# Autodesk Inventor assembly: chassis
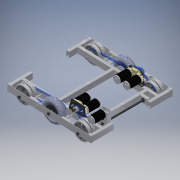
[picture p0: Inventor's stored thumbnail of the model, 180x180]
Saved by Autodesk Inventor 2016 (Build 200138000, 138)
## iProperties
Created: 2016-01-16
Part Number: chassis
Document SubType Name: Assembly
Designer: gus
Mass: 17272.6 g
Surface Area: 33201.5 cm^2
Volume: 7181.59 cm^3
Density: 2.40513 g/cm^3
Author: gus
## Documents named in this file (20)
- \\Mac\Home\Desktop\1510-stronghold-CAD\chassis\chassis.iam
- \\Mac\Home\Desktop\1510-stronghold-CAD\chassis\1x2x28.ipt
- \\Mac\Home\Desktop\1510-stronghold-CAD\chassis\1x2x19.ipt
- \\Mac\Home\Desktop\1510-stronghold-CAD\chassis\1x2x8in.ipt
- \\Mac\Home\Desktop\1510-stronghold-CAD\chassis\3 in churro.ipt
- \\Mac\Home\Desktop\1510-stronghold-CAD\chassis\side plate.ipt
- \\Mac\Home\Desktop\1510-stronghold-CAD\chassis\PneumaticWheel_am-0970-2.iam
- \\Mac\Home\Desktop\1510-stronghold-CAD\chassis\CIMple Box\CIMple Box.iam
- \\Mac\Home\Desktop\1510-stronghold-CAD\chassis\am-0736_S35-12DHE.ipt
- \\Mac\Home\Desktop\1510-stronghold-CAD\chassis\am-940a-6-HiGrip-.iam
- \\Mac\Home\Desktop\1510-stronghold-CAD\chassis\half-inch hex bolt.ipt
- \\Mac\Home\Desktop\1510-stronghold-CAD\chassis\half-inch hex nut.ipt
- \\Mac\Home\Desktop\1510-stronghold-CAD\chassis\wheel arm support.ipt
- \\Mac\Home\Desktop\1510-stronghold-CAD\roller wheels\toughbox micro\Toughbox+Nano+All+Shafts+v2-2.iam
- \\Mac\Home\Desktop\1510-stronghold-CAD\roller wheels\hex bearing.ipt
- \\Mac\Home\Desktop\1510-stronghold-CAD\chassis\chassis\Design Accelerator\Chain Drive13.iam
- \\Mac\Home\Desktop\1510-stronghold-CAD\chassis\chassis\Design Accelerator\Chain Drive14.iam
- \\Mac\Home\Desktop\1510-stronghold-CAD\chassis\chassis\Design Accelerator\Chain Drive15.iam
- \\Mac\Home\Desktop\1510-stronghold-CAD\chassis\chassis\Design Accelerator\Chain Drive16.iam
- \\Mac\Home\Desktop\1510-stronghold-CAD\chassis\chassis\Design Accelerator\Chain Drive17.iam
## Components (48 placed, 15 different names)
1. 1x2x28:1 — Mate:1, Mate:2, Flush:1, Flush:2, Mate:4, Flush:4, Flush:6, Flush:12, Flush:13, Mate:19, Rotational:7, Rotational:8, Cylindrical:25, Rotational:18, Rotational:29, Cylindrical:22, Mate:41, Flush:31, Mate:57, Mate:58
2. 1x2x19:1 — Mate:1, Flush:2, Mate:12, Mate:13, Flush:22
3. 1x2x19:2 — Mate:2, Flush:1, Mate:34, Flush:26, Flush:27, Flush:33, Mate:59, Mate:60
4. 1x2x8in:1 — Mate:8, Flush:10, Mate:13, Mate:35
5. 1x2x8in:2 — Mate:4, Flush:4, Flush:6, Mate:9, Flush:11, Mate:12, Mate:62
6. 3 in churro:1 — Mate:10, Flush:13, Flush:38
7. 3 in churro:2 — Mate:11, Flush:12, Flush:37
8. 3 in churro:3 — Flush:23, Mate:36, Flush:36
9. 3 in churro:4 — Flush:24, Mate:37, Flush:35
10. side plate:1 — Mate:8, Flush:10, Mate:21, Rotational:23, Rotational:24, Rotational:25, Mate:61
11. side plate:2 — Mate:9, Flush:11, Mate:10, Mate:11, Mate:22, Rotational:26, Rotational:27, Rotational:28, Mate:62
12. PneumaticWheel_am-0970-2:1 [sub-assembly] — Rotational:20, Flush:39, Flush:40
13. 1x2x8in:3 — Mate:19, Mate:22, Mate:53, Flush:34
14. 1x2x8in:4 — Mate:21, Mate:33, Flush:20, Flush:21, Flush:28, Mate:39, Mate:61
15. am-0736_S35-12DHE:1 — Cylindrical:2, Mate:49
16. am-0736_S35-12DHE:2 — Mate:50, Cylindrical:26
17. am-940a-6-HiGrip-:1 [sub-assembly] — Cylindrical:25, Flush:42
18. am-940a-6-HiGrip-:2 [sub-assembly] — Cylindrical:22, Flush:41
19. am-940a-6-HiGrip-:3 [sub-assembly] — Cylindrical:23, Flush:40
20. am-940a-6-HiGrip-:4 [sub-assembly] — Cylindrical:24, Flush:39
21. half-inch hex bolt:2 — Rotational:12
22. half-inch hex bolt:4 — Rotational:14
23. half-inch hex bolt:5 — Rotational:7
24. half-inch hex bolt:6 — Rotational:8
25. PneumaticWheel_am-0970-2:2 [sub-assembly] — Rotational:29, Flush:41, Flush:42
26. 1x2x28:2 — Mate:33, Flush:20, Mate:34, Flush:21, Mate:35, Flush:22, Flush:23, Flush:24, Mate:36, Mate:37, Rotational:12, Rotational:14, Cylindrical:24, Rotational:17, Rotational:20, Cylindrical:23, Mate:42, Flush:32, Mate:55, Mate:56
27. half-inch hex bolt:7 — Rotational:17
28. half-inch hex bolt:8 — Rotational:18
29. half-inch hex nut:1 — Rotational:23
30. half-inch hex nut:2 — Rotational:27
31. half-inch hex nut:3 — Rotational:25
32. half-inch hex nut:4 — Rotational:26
33. half-inch hex nut:5 — Rotational:28
34. half-inch hex nut:6 — Rotational:24
35. wheel arm support:1 — Flush:26, Flush:27, Flush:28, Mate:39, Rotational:30
36. CIMple Box:1 [sub-assembly] — Mate:41, Flush:31, Mate:50, Cylindrical:26, Mate:60
37. CIMple Box:2 [sub-assembly] — Mate:42, Flush:32, Cylindrical:2, Mate:49, Mate:59
38. Toughbox+Nano+All+Shafts+v2-2:1 [sub-assembly] — Flush:33, Mate:53, Flush:34, Mate:54
39. hex bearing:1 — Rotational:30, Mate:54
40. 3 in churro:5 — Mate:55, Flush:35
41. 3 in churro:6 — Mate:56, Flush:36
42. 3 in churro:7 — Mate:57, Flush:37
43. 3 in churro:8 — Mate:58, Flush:38
44. Chain Drive:1 [sub-assembly]
45. Chain Drive:2 [sub-assembly]
46. Chain Drive:3 [sub-assembly]
47. Chain Drive:4 [sub-assembly]
48. Chain Drive:5 [sub-assembly]
## Relationships (81: Mate 32, Flush 28, RevoluteJoint 15, CylindricalJoint 6)
- Mate:1: 1x2x28:1 ↔ 1x2x19:1
- Mate:2: 1x2x28:1 ↔ 1x2x19:2
- Flush:1: 1x2x28:1 ↔ 1x2x19:2
- Flush:2: 1x2x28:1 ↔ 1x2x19:1
- Mate:4: 1x2x28:1 ↔ 1x2x8in:2
- Flush:4: 1x2x28:1 ↔ 1x2x8in:2
- Flush:6 (101.6 mm): 1x2x28:1 ↔ 1x2x8in:2
- Mate:8: 1x2x8in:1 ↔ side plate:1
- Mate:9: 1x2x8in:2 ↔ side plate:2
- Flush:10: 1x2x8in:1 ↔ side plate:1
- Flush:11: 1x2x8in:2 ↔ side plate:2
- Mate:10: 3 in churro:1 ↔ side plate:2
- Mate:11: 3 in churro:2 ↔ side plate:2
- Mate:12 (304.8 mm): 1x2x19:1 ↔ 1x2x8in:2
- Mate:13 (304.8 mm): 1x2x19:1 ↔ 1x2x8in:1
- Flush:12 (22.225 mm): 1x2x28:1 ↔ 3 in churro:2
- Flush:13 (22.225 mm): 1x2x28:1 ↔ 3 in churro:1
- Mate:19: 1x2x28:1 ↔ 1x2x8in:3
- Mate:21: side plate:1 ↔ 1x2x8in:4
- Mate:22: side plate:2 ↔ 1x2x8in:3
- Rotational:7 [RevoluteJoint]: 1x2x28:1 ↔ half-inch hex bolt:5
- Rotational:8 [RevoluteJoint]: 1x2x28:1 ↔ half-inch hex bolt:6
- Mate:33: 1x2x8in:4 ↔ 1x2x28:2
- Flush:20: 1x2x8in:4 ↔ 1x2x28:2
- Mate:34: 1x2x19:2 ↔ 1x2x28:2
- Flush:21 (101.6 mm): 1x2x8in:4 ↔ 1x2x28:2
- Mate:35: 1x2x8in:1 ↔ 1x2x28:2
- Flush:22: 1x2x19:1 ↔ 1x2x28:2
- Flush:23 (22.225 mm): 3 in churro:3 ↔ 1x2x28:2
- Flush:24 (22.225 mm): 3 in churro:4 ↔ 1x2x28:2
- Mate:36: 3 in churro:3 ↔ 1x2x28:2
- Mate:37: 3 in churro:4 ↔ 1x2x28:2
- Rotational:12 [RevoluteJoint]: half-inch hex bolt:2 ↔ 1x2x28:2
- Rotational:14 [RevoluteJoint]: half-inch hex bolt:4 ↔ 1x2x28:2
- Cylindrical:22: 1x2x28:1 ↔ am-940a-6-HiGrip-:2
- Cylindrical:24: am-940a-6-HiGrip-:4 ↔ 1x2x28:2
- Cylindrical:23: am-940a-6-HiGrip-:3 ↔ 1x2x28:2
- Cylindrical:25: 1x2x28:1 ↔ am-940a-6-HiGrip-:1
- Rotational:17 [RevoluteJoint]: 1x2x28:2 ↔ half-inch hex bolt:7
- Rotational:18 [RevoluteJoint]: 1x2x28:1 ↔ half-inch hex bolt:8
- Rotational:20 [RevoluteJoint]: PneumaticWheel_am-0970-2:1 ↔ 1x2x28:2
- Rotational:29 [RevoluteJoint]: 1x2x28:1 ↔ PneumaticWheel_am-0970-2:2
- Rotational:23 [RevoluteJoint]: side plate:1 ↔ half-inch hex nut:1
- Rotational:24 [RevoluteJoint]: side plate:1 ↔ half-inch hex nut:6
- Rotational:25 [RevoluteJoint]: side plate:1 ↔ half-inch hex nut:3
- Rotational:26 [RevoluteJoint]: side plate:2 ↔ half-inch hex nut:4
- Rotational:27 [RevoluteJoint]: side plate:2 ↔ half-inch hex nut:2
- Rotational:28 [RevoluteJoint]: side plate:2 ↔ half-inch hex nut:5
- Flush:26: 1x2x19:2 ↔ wheel arm support:1
- Flush:27 (-10.0076 mm): 1x2x19:2 ↔ wheel arm support:1
- Flush:28: 1x2x8in:4 ↔ wheel arm support:1
- Mate:39: 1x2x8in:4 ↔ wheel arm support:1
- Mate:41: 1x2x28:1 ↔ CIMple Box:1
- Mate:42: 1x2x28:2 ↔ CIMple Box:2
- Flush:31: 1x2x28:1 ↔ CIMple Box:1
- Flush:32: 1x2x28:2 ↔ CIMple Box:2
- Cylindrical:2: am-0736_S35-12DHE:1 ↔ CIMple Box:2
- Mate:49: am-0736_S35-12DHE:1 ↔ CIMple Box:2
- Mate:50: am-0736_S35-12DHE:2 ↔ CIMple Box:1
- Cylindrical:26: am-0736_S35-12DHE:2 ↔ CIMple Box:1
- Flush:33: 1x2x19:2 ↔ Toughbox+Nano+All+Shafts+v2-2:1
- Mate:53: 1x2x8in:3 ↔ Toughbox+Nano+All+Shafts+v2-2:1
- Flush:34: 1x2x8in:3 ↔ Toughbox+Nano+All+Shafts+v2-2:1
- Rotational:30 [RevoluteJoint]: wheel arm support:1 ↔ hex bearing:1
- Mate:54: Toughbox+Nano+All+Shafts+v2-2:1 ↔ hex bearing:1
- Mate:55: 1x2x28:2 ↔ 3 in churro:5
- Flush:35: 3 in churro:4 ↔ 3 in churro:5
- Mate:56: 1x2x28:2 ↔ 3 in churro:6
- Flush:36: 3 in churro:3 ↔ 3 in churro:6
- Mate:57: 1x2x28:1 ↔ 3 in churro:7
- Flush:37: 3 in churro:2 ↔ 3 in churro:7
- Mate:58: 1x2x28:1 ↔ 3 in churro:8
- Flush:38: 3 in churro:1 ↔ 3 in churro:8
- Flush:39: PneumaticWheel_am-0970-2:1 ↔ am-940a-6-HiGrip-:4
- Flush:40: PneumaticWheel_am-0970-2:1 ↔ am-940a-6-HiGrip-:3
- Flush:41: am-940a-6-HiGrip-:2 ↔ PneumaticWheel_am-0970-2:2
- Flush:42: am-940a-6-HiGrip-:1 ↔ PneumaticWheel_am-0970-2:2
- Mate:59 (25.4 mm): 1x2x19:2 ↔ CIMple Box:2
- Mate:60 (25.4 mm): 1x2x19:2 ↔ CIMple Box:1
- Mate:61: side plate:1 ↔ 1x2x8in:4
- Mate:62: 1x2x8in:2 ↔ side plate:2
